# Autodesk Inventor assembly: Robot
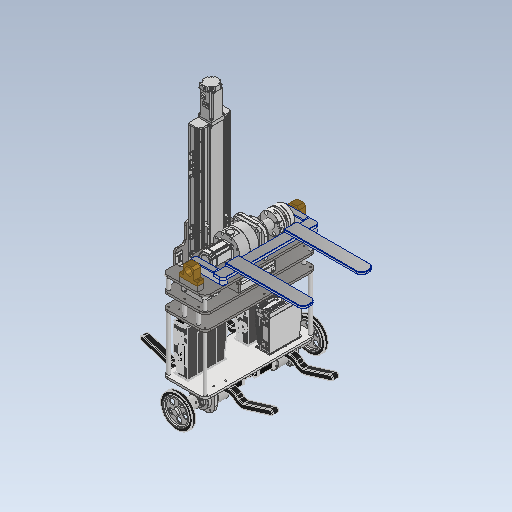
[picture p0: Inventor's stored thumbnail of the model, 512x512]
Saved by Autodesk Inventor 2025.2 (Build 292293000, 293)
## iProperties
Created: 2025-02-20
Part Number: Robot
Document SubType Name: Assembly
Designer: Sergio Quintero
Author: Sergio Quintero
## Documents named in this file (34)
- C:\Users\Sergio Quintero\OneDrive - Universidad Nacional de Colombia\Keio University\Thesis\CAD\Ball_screw\Robot.iam
- C:\Users\Sergio Quintero\OneDrive - Universidad Nacional de Colombia\Keio University\Thesis\CAD\Ball_screw\Bottom_plate.ipt
- C:\Users\Sergio Quintero\OneDrive - Universidad Nacional de Colombia\Keio University\Thesis\CAD\Ball_screw\Top_plate.ipt
- C:\Users\Sergio Quintero\OneDrive - Universidad Nacional de Colombia\Keio University\Thesis\CAD\Ball_screw\Structure_bar.ipt
- C:\Users\Sergio Quintero\OneDrive - Universidad Nacional de Colombia\Keio University\Thesis\CAD\Ball_screw\Pillow_support.ipt
- C:\Users\Sergio Quintero\OneDrive - Universidad Nacional de Colombia\Keio University\Thesis\CAD\Ball_screw\Pillow_block.ipt
- C:\Users\Sergio Quintero\OneDrive - Universidad Nacional de Colombia\Keio University\Thesis\CAD\Ball_screw\Gear_support.ipt
- C:\Users\Sergio Quintero\OneDrive - Universidad Nacional de Colombia\Keio University\Thesis\CAD\Ball_screw\HPG-32A-33-J2NELA.iam
- C:\Users\Sergio Quintero\OneDrive - Universidad Nacional de Colombia\Keio University\Thesis\CAD\Ball_screw\SFC-090SA2-25B-40B.ipt
- C:\Users\Sergio Quintero\OneDrive - Universidad Nacional de Colombia\Keio University\Thesis\CAD\Ball_screw\Fork.ipt
- C:\Users\Sergio Quintero\OneDrive - Universidad Nacional de Colombia\Keio University\Thesis\CAD\Ball_screw\Gear_support_wheel.ipt
- C:\Users\Sergio Quintero\OneDrive - Universidad Nacional de Colombia\Keio University\Thesis\CAD\Ball_screw\HPG-20A-11-J6GDK.iam
- C:\Users\Sergio Quintero\OneDrive - Universidad Nacional de Colombia\Keio University\Thesis\CAD\Ball_screw\MRG-50-25-25.ipt
- C:\Users\Sergio Quintero\OneDrive - Universidad Nacional de Colombia\Keio University\Thesis\CAD\Ball_screw\Wheel.ipt
- C:\Users\Sergio Quintero\OneDrive - Universidad Nacional de Colombia\Keio University\Thesis\CAD\Ball_screw\R88M_K40030S.ipt
- C:\Users\Sergio Quintero\OneDrive - Universidad Nacional de Colombia\Keio University\Thesis\CAD\Ball_screw\R88M_1M40030S_S2.ipt
- C:\Users\Sergio Quintero\OneDrive - Universidad Nacional de Colombia\Keio University\Thesis\CAD\Ball_screw\Robot_support.ipt
- C:\Users\Sergio Quintero\OneDrive - Universidad Nacional de Colombia\Keio University\Thesis\CAD\Ball_screw\R88D_1SN04L_ECT\R88D_1SN04L_ECT.iam
- C:\Users\Sergio Quintero\OneDrive - Universidad Nacional de Colombia\Keio University\Thesis\CAD\Ball_screw\R88D_KN04L_ECT\R88D_KN04L_ECT.iam
- C:\Users\Sergio Quintero\OneDrive - Universidad Nacional de Colombia\Keio University\Thesis\CAD\Ball_screw\Mid_structure_bar.ipt
- C:\Users\Sergio Quintero\OneDrive - Universidad Nacional de Colombia\Keio University\Thesis\CAD\Ball_screw\mr-j4-40ab.iam
- C:\Users\Sergio Quintero\OneDrive - Universidad Nacional de Colombia\Keio University\Thesis\CAD\Ball_screw\Current_plate.ipt
- C:\Users\Sergio Quintero\OneDrive - Universidad Nacional de Colombia\Keio University\Thesis\CAD\Ball_screw\Support_bar.ipt
- C:\Users\Sergio Quintero\OneDrive - Universidad Nacional de Colombia\Keio University\Thesis\CAD\Ball_screw\Support_plate.ipt
- C:\Users\Sergio Quintero\OneDrive - Universidad Nacional de Colombia\Keio University\Thesis\CAD\Ball_screw\Rubber_feet.ipt
- C:\Users\Sergio Quintero\OneDrive - Universidad Nacional de Colombia\Keio University\Thesis\CAD\Ball_screw\Support_lift.ipt
- C:\Users\Sergio Quintero\OneDrive - Universidad Nacional de Colombia\Keio University\Thesis\CAD\Ball_screw\AIS2024\ETH2-17-L5-350-BC-M40B-C6N5L(350).iam
- C:\Users\Sergio Quintero\OneDrive - Universidad Nacional de Colombia\Keio University\Thesis\CAD\Ball_screw\Mobile.ipt
- C:\Users\Sergio Quintero\OneDrive - Universidad Nacional de Colombia\Keio University\Thesis\CAD\Ball_screw\Horizontal_support.ipt
- C:\Users\Sergio Quintero\OneDrive - Universidad Nacional de Colombia\Keio University\Thesis\CAD\Ball_screw\L_Bracket.ipt
- C:\Users\Sergio Quintero\OneDrive - Universidad Nacional de Colombia\Keio University\Thesis\CAD\Ball_screw\Angle_fork.ipt
- C:\Users\Sergio Quintero\OneDrive - Universidad Nacional de Colombia\Keio University\Thesis\CAD\Ball_screw\Lift_adaptor.ipt
- C:\Users\Sergio Quintero\OneDrive - Universidad Nacional de Colombia\Keio University\Thesis\CAD\Ball_screw\Support_driver.ipt
- C:\Users\Sergio Quintero\OneDrive - Universidad Nacional de Colombia\Keio University\Thesis\CAD\Ball_screw\S8FS_G01524C\S8FS_G01524C.iam
## Components (58 placed, 33 different names)
1. Bottom_plate:1 — Rigid:1, Rigid:2, Rigid:3, Rigid:4, Rigid:13, Rigid:14, Angle:1, Rigid:23, Rigid:24, Rigid:25, Rigid:26, Rigid:27, Rigid:28, Rigid:29, Rigid:37
2. Top_plate:1 — Rigid:6, Rigid:8, Rigid:10, Rigid:77
3. Structure_bar:1 — Rigid:4
4. Structure_bar:2 — Rigid:3
5. Structure_bar:3 — Rigid:2
6. Structure_bar:4 — Rigid:1
7. Pillow_support:1 — Rigid:6, Rigid:7
8. Pillow_block:1 — Rigid:7
9. Pillow_block:2 — Rigid:9, Rotational:1
10. Pillow_support:2 — Rigid:8, Rigid:9
11. Gear_support:1 — Rigid:10, Rigid:11
12. HPG-32A-33-J2NELA:1 [sub-assembly] — Rigid:11, Rigid:12, Rigid:21
13. SFC-090SA2-25B-40B:1 — Rigid:12
14. Fork:1 — Rotational:1
15. Gear_support_wheel:1 — Rigid:14, Rigid:15
16. Gear_support_wheel:2 — Rigid:13, Rigid:16
17. HPG-20A-11-J6GDK:1 [sub-assembly] — Rigid:15, Rigid:18, Rotational:2
18. HPG-20A-11-J6GDK:2 [sub-assembly] — Rigid:16, Rigid:17, Rigid:22
19. MRG-50-25-25:1 — Rigid:17, Rigid:20
20. MRG-50-25-25:2 — Rigid:18, Rigid:19
21. Wheel:1 — Rigid:20
22. Wheel:2 — Rigid:19, Tangent:1
23. R88M_K40030S:1 — Rigid:21
24. R88M_1M40030S_S2:1 — Rigid:22
25. R88M_1M40030S_S2:2 — Rotational:2
26. Robot_support:1 — Rigid:23
27. Robot_support:2 — Rigid:24
28. Robot_support:3 — Rigid:25
29. Robot_support:4 — Rigid:26
30. R88D_1SN04L_ECT:1 [sub-assembly] — Rigid:27
31. R88D_1SN04L_ECT:2 [sub-assembly] — Rigid:28
32. R88D_KN04L_ECT:1 [sub-assembly] — Rigid:29
33. Mid_structure_bar:1 — Rigid:62, Rigid:81
34. Mid_structure_bar:2 — Rigid:61, Rigid:80
35. Mid_structure_bar:3 — Rigid:63, Rigid:78
36. Mid_structure_bar:4 — Rigid:64, Rigid:79
37. Current_plate:1 — Rigid:37, Rigid:43, Rigid:44, Rigid:45, Rigid:46, Rigid:47
38. mr-j4-40ab:1 [sub-assembly] — Rigid:71
39. Support_bar:1 — Rigid:43
40. Support_bar:2 — Rigid:44
41. Support_bar:3 — Rigid:45
42. Support_bar:4 — Rigid:46
43. Support_plate:1 — Rigid:47, Rigid:61, Rigid:62, Rigid:63, Rigid:64, Rotational:3, Rigid:70, Rigid:71, Rigid:75, Rigid:82
44. Support_lift:1 — Rigid:69
45. ETH2-17-L5-350-BC-M40B-C6N5L(350):1 [sub-assembly] — Slider:1, Rigid:69
46. Mobile:1 — Slider:1, Rigid:74
47. Horizontal_support:1 — Rotational:3, Rigid:72
48. Horizontal_support:2 — Rigid:70, Rigid:73
49. L_Bracket:1 — Rigid:72
50. L_Bracket:2 — Rigid:73
51. Angle_fork:1 — Rotational:4, Rigid:77
52. Lift_adaptor:1 — Rigid:74, Rotational:4
53. Support_driver:1 — Rigid:75
54. S8FS_G01524C:1 [sub-assembly] — Rigid:82
55. Rubber_feet:1 — Rigid:80
56. Rubber_feet:2 — Rigid:81
57. Rubber_feet:3 — Rigid:78
58. Rubber_feet:4 — Rigid:79
## Relationships (58: WeldJoint 51, RevoluteJoint 4, Angle 1, Tangent 1, TranslationJoint 1)
- Rigid:1 [WeldJoint]: Bottom_plate:1 ↔ Structure_bar:4
- Rigid:2 [WeldJoint]: Bottom_plate:1 ↔ Structure_bar:3
- Rigid:3 [WeldJoint]: Bottom_plate:1 ↔ Structure_bar:2
- Rigid:4 [WeldJoint]: Bottom_plate:1 ↔ Structure_bar:1
- Rigid:6 [WeldJoint]: Top_plate:1 ↔ Pillow_support:1
- Rigid:7 [WeldJoint]: Pillow_support:1 ↔ Pillow_block:1
- Rigid:8 [WeldJoint]: Top_plate:1 ↔ Pillow_support:2
- Rigid:9 [WeldJoint]: Pillow_block:2 ↔ Pillow_support:2
- Rigid:10 [WeldJoint]: Top_plate:1 ↔ Gear_support:1
- Rigid:11 [WeldJoint]: Gear_support:1 ↔ HPG-32A-33-J2NELA:1
- Rigid:12 [WeldJoint] (50 mm): HPG-32A-33-J2NELA:1 ↔ SFC-090SA2-25B-40B:1
- Rotational:1 [RevoluteJoint] (5 mm): Pillow_block:2 ↔ Fork:1
- Rigid:13 [WeldJoint]: Bottom_plate:1 ↔ Gear_support_wheel:2
- Rigid:14 [WeldJoint]: Bottom_plate:1 ↔ Gear_support_wheel:1
- Rigid:15 [WeldJoint]: Gear_support_wheel:1 ↔ HPG-20A-11-J6GDK:1
- Rigid:16 [WeldJoint]: Gear_support_wheel:2 ↔ HPG-20A-11-J6GDK:2
- Rigid:17 [WeldJoint] (15 mm): HPG-20A-11-J6GDK:2 ↔ MRG-50-25-25:1
- Rigid:18 [WeldJoint] (15 mm): HPG-20A-11-J6GDK:1 ↔ MRG-50-25-25:2
- Rigid:19 [WeldJoint] (3 mm): MRG-50-25-25:2 ↔ Wheel:2
- Rigid:20 [WeldJoint] (3 mm): MRG-50-25-25:1 ↔ Wheel:1
- Rigid:21 [WeldJoint]: HPG-32A-33-J2NELA:1 ↔ R88M_K40030S:1
- Rigid:22 [WeldJoint]: HPG-20A-11-J6GDK:2 ↔ R88M_1M40030S_S2:1
- Rotational:2 [RevoluteJoint]: HPG-20A-11-J6GDK:1 ↔ R88M_1M40030S_S2:2
- Angle:1 (0 deg): Bottom_plate:1
- Tangent:1: Wheel:2
- Rigid:23 [WeldJoint]: Bottom_plate:1 ↔ Robot_support:1
- Rigid:24 [WeldJoint]: Bottom_plate:1 ↔ Robot_support:2
- Rigid:25 [WeldJoint]: Bottom_plate:1 ↔ Robot_support:3
- Rigid:26 [WeldJoint]: Bottom_plate:1 ↔ Robot_support:4
- Rigid:27 [WeldJoint]: Bottom_plate:1 ↔ R88D_1SN04L_ECT:1
- Rigid:28 [WeldJoint]: Bottom_plate:1 ↔ R88D_1SN04L_ECT:2
- Rigid:29 [WeldJoint]: Bottom_plate:1 ↔ R88D_KN04L_ECT:1
- Rigid:37 [WeldJoint] (260 mm): Bottom_plate:1 ↔ Current_plate:1
- Rigid:43 [WeldJoint]: Current_plate:1 ↔ Support_bar:1
- Rigid:44 [WeldJoint]: Current_plate:1 ↔ Support_bar:2
- Rigid:45 [WeldJoint]: Current_plate:1 ↔ Support_bar:3
- Rigid:46 [WeldJoint]: Current_plate:1 ↔ Support_bar:4
- Rigid:47 [WeldJoint] (60 mm): Current_plate:1 ↔ Support_plate:1
- Rigid:61 [WeldJoint]: Mid_structure_bar:2 ↔ Support_plate:1
- Rigid:62 [WeldJoint]: Mid_structure_bar:1 ↔ Support_plate:1
- Rigid:63 [WeldJoint]: Mid_structure_bar:3 ↔ Support_plate:1
- Rigid:64 [WeldJoint]: Mid_structure_bar:4 ↔ Support_plate:1
- Slider:1 [TranslationJoint] (2.252 mm): ETH2-17-L5-350-BC-M40B-C6N5L(350):1 ↔ Mobile:1
- Rigid:69 [WeldJoint]: Support_lift:1 ↔ ETH2-17-L5-350-BC-M40B-C6N5L(350):1
- Rotational:3 [RevoluteJoint]: Support_plate:1 ↔ Horizontal_support:1
- Rigid:70 [WeldJoint]: Support_plate:1 ↔ Horizontal_support:2
- Rigid:71 [WeldJoint] (-5 mm): mr-j4-40ab:1 ↔ Support_plate:1
- Rigid:72 [WeldJoint] (-10 mm): Horizontal_support:1 ↔ L_Bracket:1
- Rigid:73 [WeldJoint] (-10 mm): Horizontal_support:2 ↔ L_Bracket:2
- Rigid:74 [WeldJoint]: Mobile:1 ↔ Lift_adaptor:1
- Rotational:4 [RevoluteJoint]: Angle_fork:1 ↔ Lift_adaptor:1
- Rigid:75 [WeldJoint]: Support_plate:1 ↔ Support_driver:1
- Rigid:77 [WeldJoint]: Top_plate:1 ↔ Angle_fork:1
- Rigid:78 [WeldJoint]: Mid_structure_bar:3 ↔ Rubber_feet:3
- Rigid:79 [WeldJoint]: Mid_structure_bar:4 ↔ Rubber_feet:4
- Rigid:80 [WeldJoint]: Mid_structure_bar:2 ↔ Rubber_feet:1
- Rigid:81 [WeldJoint]: Mid_structure_bar:1 ↔ Rubber_feet:2
- Rigid:82 [WeldJoint] (-40 mm): Support_plate:1 ↔ S8FS_G01524C:1
